# Autodesk Inventor assembly: Trasmissione cinghie - Taglio
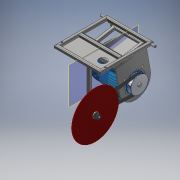
[picture p0: Inventor's stored thumbnail of the model, 180x180]
Saved by Autodesk Inventor 2018 (Build 220112000, 112)
## iProperties
Created: 2020-06-04
Part Number: Trasmissione cinghie - Taglio
Material: Generico
Document SubType Name: Assembly
Designer: Francesco
Mass: 11579.7 g
Surface Area: 9613.4 cm^2
Volume: 5451 cm^3
Density: 2.12433 g/cm^3
Author: Francesco
## Documents named in this file (17)
- C:\Users\Francesco\no-brim\Meccanica\Progetto Inventor no-brim\Assiemi\Trasmissione cinghie - Taglio.iam
- C:\Users\Francesco\no-brim\Meccanica\Progetto Inventor no-brim\Parti\Puleggia maggiore.ipt
- C:\Users\Francesco\no-brim\Meccanica\Progetto Inventor no-brim\Parti\Puleggia minore.ipt
- C:\Users\Francesco\no-brim\Meccanica\Progetto Inventor no-brim\Parti\Cinghia.ipt
- C:\Users\Francesco\no-brim\Meccanica\Progetto Inventor no-brim\Parti\Sega Circolare 300 mm.ipt
- C:\Users\Francesco\no-brim\Meccanica\Progetto Inventor no-brim\Parti\Motorredutor Bonfiglioli .iam
- C:\Users\Francesco\no-brim\Meccanica\Progetto Inventor no-brim\Parti\Lamiera supporto motore.ipt
- C:\Users\Francesco\no-brim\Meccanica\Progetto Inventor no-brim\Assiemi\Telaietto trasmissione - Taglio.iam
- C:\Users\Francesco\no-brim\Meccanica\Progetto Inventor no-brim\Parti\Distanziale lama.ipt
- C:\Users\Francesco\no-brim\Meccanica\Progetto Inventor no-brim\Unificati\it-IT\UNI 8836\UNI 8836 - 21,4 x 38 - 4,6.ipt
- C:\Users\Francesco\no-brim\Meccanica\Progetto Inventor no-brim\Unificati\it-IT\ISO 7043\ISO 7043 - M16 - ISO.ipt
- C:\Users\Francesco\no-brim\Meccanica\Progetto Inventor no-brim\Unificati\it-IT\SKF B - angular contact\SKF B7204 BE.ipt
- C:\Users\Francesco\no-brim\Meccanica\Progetto Inventor no-brim\Parti\Porta cuscinetto puleggia operatrice.ipt
- C:\Users\Francesco\no-brim\Meccanica\Progetto Inventor no-brim\Parti\Lamiera telaietto.ipt
- C:\Users\Francesco\no-brim\Meccanica\Progetto Inventor no-brim\Unificati\it-IT\DIN 976-1 B\DIN 976-1 - M8 x 70 - B.ipt
- C:\Users\Francesco\no-brim\Meccanica\Progetto Inventor no-brim\Unificati\it-IT\UNI 5721\UN 5721 - M8 - 1,25.ipt
- C:\Users\Francesco\no-brim\Meccanica\Progetto Inventor no-brim\Unificati\it-IT\ISO 4035(2)\ISO 4035 - M8 - ISO.ipt
## Components (16 placed, 16 different names)
1. Puleggia maggiore:1 — Allineato:1, Coincidente:2, Coincidente:3, Coincidente:11, Angolo:1, Coincidente:15
2. Puleggia minore:1 — Allineato:1, Coincidente:1, Coincidente:4, Coincidente:17, Coincidente:18, Coincidente:19, Coincidente:21, Coincidente:23, Coincidente:27, Coincidente:28
3. Cinghia:1 — Coincidente:1, Coincidente:2, Coincidente:3
4. Sega Circolare 300 mm:1 — Coincidente:4, Coincidente:20, Coincidente:22
5. Lamiera supporto motore:1 — Coincidente:11, Angolo:1, Coincidente:13, Coincidente:14, Angolo:2, Coincidente:16, Allineato:6, Allineato:7, Coincidente:33, Coincidente:36
6. Motorredutor Bonfiglioli :1 [sub-assembly] — Coincidente:13, Coincidente:14, Angolo:2, Coincidente:15
7. Telaietto trasmissione:1 [sub-assembly] — Allineato:5, Coincidente:16, Allineato:6, Allineato:7, Coincidente:17, Coincidente:29, Coincidente:30, Coincidente:31, Coincidente:38, Angolo:3
8. Distanziale lama:1 — Coincidente:18, Coincidente:19, Coincidente:20
9. UNI 8836 21,4 x 38:1 — Coincidente:21, Coincidente:22, Coincidente:24
10. ISO 7043 M16:1 — Coincidente:23, Coincidente:24
11. SKF B- Contatto angolare SKF B7204 BE:1 — Coincidente:25, Coincidente:26, Coincidente:27
12. Porta cuscinetto puleggia operatrice:1 — Coincidente:25, Coincidente:26, Coincidente:28, Coincidente:29
13. Lamiera telaietto:1 — Coincidente:30, Coincidente:31, Coincidente:32, Coincidente:34
14. DIN 976-1 B M8 x 70:1 — Coincidente:33, Coincidente:34, Coincidente:35, Coincidente:37
15. UNI 5721 M8:1 — Coincidente:35, Coincidente:36
16. ISO 4035 M8:1 — Coincidente:37, Coincidente:38, Angolo:3
## Relationships (38: Mate 31, Flush 4, Angle 3)
- Allineato:1 [Flush]: Puleggia maggiore:1 ↔ Puleggia minore:1
- Coincidente:1 [Mate]: Puleggia minore:1 ↔ Cinghia:1
- Coincidente:2 [Mate]: Puleggia maggiore:1 ↔ Cinghia:1
- Coincidente:3 [Mate] (1.5 mm): Puleggia maggiore:1 ↔ Cinghia:1
- Coincidente:4 [Mate]: Puleggia minore:1 ↔ Sega Circolare 300 mm:1
- Coincidente:11 [Mate]: Puleggia maggiore:1 ↔ Lamiera supporto motore:1
- Angolo:1 [Angle] (0 deg): Puleggia maggiore:1 ↔ Lamiera supporto motore:1
- Coincidente:13 [Mate]: Lamiera supporto motore:1 ↔ Motorredutor Bonfiglioli :1
- Coincidente:14 [Mate]: Lamiera supporto motore:1 ↔ Motorredutor Bonfiglioli :1
- Angolo:2 [Angle] (-90 deg): Lamiera supporto motore:1 ↔ Motorredutor Bonfiglioli :1
- Coincidente:15 [Mate]: Puleggia maggiore:1 ↔ Motorredutor Bonfiglioli :1
- Allineato:5 [Flush] (-150 mm): Telaietto trasmissione:1
- Coincidente:16 [Mate]: Lamiera supporto motore:1 ↔ Telaietto trasmissione:1
- Allineato:6 [Flush]: Lamiera supporto motore:1 ↔ Telaietto trasmissione:1
- Allineato:7 [Flush]: Lamiera supporto motore:1 ↔ Telaietto trasmissione:1
- Coincidente:17 [Mate] (210 mm): Puleggia minore:1 ↔ Telaietto trasmissione:1
- Coincidente:18 [Mate]: Puleggia minore:1 ↔ Distanziale lama:1
- Coincidente:19 [Mate]: Puleggia minore:1 ↔ Distanziale lama:1
- Coincidente:20 [Mate]: Sega Circolare 300 mm:1 ↔ Distanziale lama:1
- Coincidente:21 [Mate]: Puleggia minore:1 ↔ UNI 8836 21,4 x 38:1
- Coincidente:22 [Mate]: Sega Circolare 300 mm:1 ↔ UNI 8836 21,4 x 38:1
- Coincidente:23 [Mate]: Puleggia minore:1 ↔ ISO 7043 M16:1
- Coincidente:24 [Mate]: UNI 8836 21,4 x 38:1 ↔ ISO 7043 M16:1
- Coincidente:25 [Mate]: SKF B- Contatto angolare SKF B7204 BE:1 ↔ Porta cuscinetto puleggia operatrice:1
- Coincidente:26 [Mate]: SKF B- Contatto angolare SKF B7204 BE:1 ↔ Porta cuscinetto puleggia operatrice:1
- Coincidente:27 [Mate]: Puleggia minore:1 ↔ SKF B- Contatto angolare SKF B7204 BE:1
- Coincidente:28 [Mate] (5 mm): Puleggia minore:1 ↔ Porta cuscinetto puleggia operatrice:1
- Coincidente:29 [Mate]: Telaietto trasmissione:1 ↔ Porta cuscinetto puleggia operatrice:1
- Coincidente:30 [Mate]: Telaietto trasmissione:1 ↔ Lamiera telaietto:1
- Coincidente:31 [Mate]: Telaietto trasmissione:1 ↔ Lamiera telaietto:1
- Coincidente:32 [Mate]: Lamiera telaietto:1
- Coincidente:33 [Mate]: Lamiera supporto motore:1 ↔ DIN 976-1 B M8 x 70:1
- Coincidente:34 [Mate]: Lamiera telaietto:1 ↔ DIN 976-1 B M8 x 70:1
- Coincidente:35 [Mate]: DIN 976-1 B M8 x 70:1 ↔ UNI 5721 M8:1
- Coincidente:36 [Mate]: Lamiera supporto motore:1 ↔ UNI 5721 M8:1
- Coincidente:37 [Mate]: DIN 976-1 B M8 x 70:1 ↔ ISO 4035 M8:1
- Coincidente:38 [Mate]: Telaietto trasmissione:1 ↔ ISO 4035 M8:1
- Angolo:3 [Angle] (0 deg): Telaietto trasmissione:1 ↔ ISO 4035 M8:1
